# Autodesk Inventor assembly: worm_gear
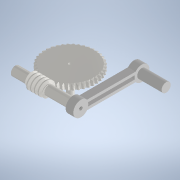
[picture p0: Inventor's stored thumbnail of the model, 180x180]
Saved by Autodesk Inventor 2020 (Build 240168000, 168)
## iProperties
Created: 2020-05-17
Part Number: worm_gear
Document SubType Name: Assembly
Designer: Hesekiel
Author: Hesekiel
## Documents named in this file (4)
- C:\Users\Hesekiel\Documents\Inventor\Uchwyt Aktywny Teleskopu\worm_gear.iam
- C:\Users\Hesekiel\Documents\Inventor\Uchwyt Aktywny Teleskopu\worm_gear\Design Accelerator\Worm Gears1.iam
- C:\Users\Hesekiel\Desktop\Equatorial-Mount-MUM\Mechanika\Mechanizm elewacji Filip\CAD\ramię_korby.ipt
- C:\Users\Hesekiel\Desktop\Equatorial-Mount-MUM\Mechanika\Mechanizm elewacji Filip\CAD\rączka_korby.ipt
## Components (3 placed, 3 different names)
1. Worm Gears:1 [sub-assembly] — Rigid:1
2. ramię_korby:1 — Rigid:1, Rigid:2
3. rączka_korby:1 — Rigid:2
## Relationships (2: WeldJoint 2)
- Rigid:1 [WeldJoint]: Worm Gears:1 ↔ ramię_korby:1
- Rigid:2 [WeldJoint]: ramię_korby:1 ↔ rączka_korby:1
